# Autodesk Inventor assembly: Base_Roulante_Ammovible
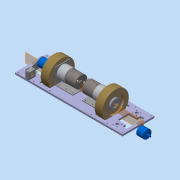
[picture p0: Inventor's stored thumbnail of the model, 180x180]
Saved by Autodesk Inventor 2016 (Build 200138000, 138)
## iProperties
Created: 2012-09-17
Part Number: Base_Roulante_Ammovible
Document SubType Name: Assembly
Designer: Aegir
Author: Aegir
## Documents named in this file (10)
- C:\Users\Aegir\Documents\robotik 2017\git\base roulante_v2\conception\Base_Roulante_Ammovible.iam
- C:\Users\Aegir\Documents\robotik 2017\git\base roulante_v2\conception\Base_Moteur.ipt
- C:\Users\Aegir\Documents\robotik 2017\git\base roulante_v2\conception\Ammortisseurv2.iam
- C:\Users\Aegir\Documents\robotik 2017\git\base roulante_v2\conception\ensemble_moteur.iam
- C:\Users\Aegir\Documents\robotik 2017\git\base roulante_v2\conception\moyeux_expansible.ipt
- C:\Users\Aegir\Documents\robotik 2017\git\base roulante_v2\conception\Colson_Wheel_3in_x_7_8in.ipt
- C:\Users\Aegir\Documents\robotik 2017\git\base roulante_v2\conception\palier_roulement_bras.ipt
- C:\Users\Aegir\Documents\Inventor\Content Center Files\R2016\fr-FR\ISO 2795  C\ISO 2795 - 5 x 9 x 8C.ipt
- C:\Users\Aegir\Documents\robotik 2017\git\base roulante_v2\conception\bras_codeur.ipt
- C:\Users\Aegir\Documents\robotik 2017\git\base roulante_v2\conception\crochet.ipt
## Components (14 placed, 10 different names)
1. Base_Moteur.1 — Placage:3, Placage:4, Affleurement:2, Affleurement:3, Placage:5, Placage:14, Affleurement:11, Placage:18, Affleurement:13, Angle:2
2. Ammortisseurv2.1 [sub-assembly] — Placage:16, Placage:24, Placage:25
3. Ammortisseurv2.2 [sub-assembly]
4. ensemble_moteur:1 [sub-assembly] — Placage:3, Affleurement:2, Placage:5, Placage:6, Placage:7, Affleurement:5
5. ensemble_moteur:2 [sub-assembly] — Placage:4, Affleurement:3, Placage:6, Placage:8, Affleurement:4
6. moyeux_expansible:1 — Placage:7, Affleurement:5, Affleurement:6, Placage:10
7. moyeux_expansible:2 — Placage:8, Affleurement:4, Placage:9, Affleurement:7
8. Colson_Wheel_3in_x_7_8in:1 — Placage:9, Affleurement:7, Placage:16, Placage:19
9. Colson_Wheel_3in_x_7_8in:2 — Affleurement:6, Placage:10, Placage:11
10. palier_roulement_bras:1 — Placage:14, Affleurement:11, Placage:21, Affleurement:14, Placage:23
11. ISO 2795 (Cylindriques) 5 x 9 x 8:1 — Placage:21, Affleurement:14, Placage:22
12. crochet:1
13. crochet:2 — Placage:18, Affleurement:13
14. bras_codeur:1 — Placage:22, Placage:23, Placage:24, Placage:25
## Relationships (29: Mate 19, Flush 9, Angle 1)
- Placage:3 [Mate]: Base_Moteur.1 ↔ ensemble_moteur:1
- Placage:4 [Mate]: Base_Moteur.1 ↔ ensemble_moteur:2
- Affleurement:2 [Flush]: Base_Moteur.1 ↔ ensemble_moteur:1
- Affleurement:3 [Flush]: Base_Moteur.1 ↔ ensemble_moteur:2
- Placage:5 [Mate] (-46 mm): Base_Moteur.1 ↔ ensemble_moteur:1
- Placage:6 [Mate]: ensemble_moteur:1 ↔ ensemble_moteur:2
- Placage:7 [Mate]: ensemble_moteur:1 ↔ moyeux_expansible:1
- Placage:8 [Mate]: ensemble_moteur:2 ↔ moyeux_expansible:2
- Affleurement:4 [Flush]: ensemble_moteur:2 ↔ moyeux_expansible:2
- Affleurement:5 [Flush]: ensemble_moteur:1 ↔ moyeux_expansible:1
- Placage:9 [Mate]: moyeux_expansible:2 ↔ Colson_Wheel_3in_x_7_8in:1
- Affleurement:6 [Flush] (-4 mm): moyeux_expansible:1 ↔ Colson_Wheel_3in_x_7_8in:2
- Placage:10 [Mate]: moyeux_expansible:1 ↔ Colson_Wheel_3in_x_7_8in:2
- Placage:11 [Mate]: Colson_Wheel_3in_x_7_8in:2
- Affleurement:7 [Flush] (4 mm): moyeux_expansible:2 ↔ Colson_Wheel_3in_x_7_8in:1
- Placage:14 [Mate]: Base_Moteur.1 ↔ palier_roulement_bras:1
- Affleurement:11 [Flush]: Base_Moteur.1 ↔ palier_roulement_bras:1
- Placage:16 [Mate]: Ammortisseurv2.1 ↔ Colson_Wheel_3in_x_7_8in:1
- Placage:18 [Mate]: Base_Moteur.1 ↔ crochet:2
- Affleurement:13 [Flush]: Base_Moteur.1 ↔ crochet:2
- Placage:19 [Mate]: Colson_Wheel_3in_x_7_8in:1
- Placage:20 [Mate]
- Angle:2 (180 deg): Base_Moteur.1
- Placage:21 [Mate]: palier_roulement_bras:1 ↔ ISO 2795 (Cylindriques) 5 x 9 x 8:1
- Affleurement:14 [Flush]: palier_roulement_bras:1 ↔ ISO 2795 (Cylindriques) 5 x 9 x 8:1
- Placage:22 [Mate]: ISO 2795 (Cylindriques) 5 x 9 x 8:1 ↔ bras_codeur:1
- Placage:23 [Mate]: palier_roulement_bras:1 ↔ bras_codeur:1
- Placage:24 [Mate]: Ammortisseurv2.1 ↔ bras_codeur:1
- Placage:25 [Mate]: Ammortisseurv2.1 ↔ bras_codeur:1
